# Autodesk Inventor assembly: Head
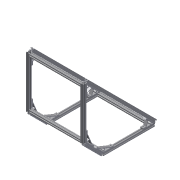
[picture p0: Inventor's stored thumbnail of the model, 180x180]
Saved by Autodesk Inventor 2014 SP1 (Build 180222100, 222)
## iProperties
Created: 2015-02-11
Part Number: Head
Document SubType Name: Assembly
Designer: Simen
Author: Simen
## Documents named in this file (6)
- C:\Users\Simen\Documents\git\Eit\skjellet\Head.iam
- C:\Users\Simen\Documents\git\Eit\skjellet\KHFS5_2020_350.ipt
- C:\Users\Simen\Documents\git\Eit\skjellet\HBL45TS6hbl45ts6.ipt
- C:\Users\Simen\Documents\git\Eit\skjellet\KHFS5_2020_660.ipt
- C:\Users\Simen\Documents\git\Eit\skjellet\HBL135TS6.iam
- C:\Users\Simen\Documents\git\Eit\skjellet\KHFS5_2020_165.ipt
## Components (20 placed, 3 different names)
1. HBL45TS6hbl45ts6:1 — Mate:1, Flush:1, Mate:2, Mate:23
2. KHFS5-2020-4000:1 — Mate:1, Flush:1, Mate:2, Flush:2, Angle:1, Mate:3, Mate:6, Flush:5, Mate:7, Mate:24, Flush:13, Flush:14, Mate:30, Flush:23, Flush:24
3. KHFS5-2020-4000:2 — Flush:2, Angle:1, Mate:3, Mate:21, Mate:22, Flush:12, Mate:23, Flush:22
4. HBL135TS6:1 [sub-assembly] — Mate:6, Flush:5, Mate:7
5. KHFS5-2020-4000:3 — Mate:24, Flush:13, Flush:14, Mate:25, Flush:15, Flush:16
6. KHFS5-2020-4000:4 — Mate:26, Flush:17, Flush:18, Mate:27, Flush:19, Flush:20
7. KHFS5-2020-4000:7 — Mate:25, Flush:15, Flush:16
8. HBL45TS6hbl45ts6:2
9. HBL135TS6:2 [sub-assembly] — Mate:31, Flush:27
10. KHFS5-2020-4000:8 — Mate:27, Flush:19, Flush:20, Flush:21
11. HBL45TS6hbl45ts6:3 — Mate:28
12. HBL135TS6:3 [sub-assembly] — Mate:32
13. KHFS5-2020-4000:9 — Mate:22, Flush:12, Mate:26, Flush:17, Flush:18, Mate:29, Flush:25, Flush:26
14. HBL45TS6hbl45ts6:4 — Mate:21
15. HBL135TS6:4 [sub-assembly] — Mate:33, Flush:28
16. KHFS5-2020-4000:10 — Flush:21, Mate:28, Flush:22
17. KHFS5-2020-4000:11 — Mate:30, Flush:23, Flush:24
18. KHFS5-2020-4000:12 — Mate:29, Flush:25, Flush:26
19. KHFS5-2020-4000:13 — Mate:31, Flush:27, Mate:32, Flush:29
20. KHFS5-2020-4000:14 — Mate:33, Flush:28, Flush:29
## Relationships (58: Mate 30, Flush 27, Angle 1)
- Mate:1: HBL45TS6hbl45ts6:1 ↔ KHFS5-2020-4000:1
- Flush:1: HBL45TS6hbl45ts6:1 ↔ KHFS5-2020-4000:1
- Mate:2: HBL45TS6hbl45ts6:1 ↔ KHFS5-2020-4000:1
- Flush:2: KHFS5-2020-4000:1 ↔ KHFS5-2020-4000:2
- Angle:1 (-45 deg): KHFS5-2020-4000:1 ↔ KHFS5-2020-4000:2
- Mate:3: KHFS5-2020-4000:1 ↔ KHFS5-2020-4000:2
- Mate:6: KHFS5-2020-4000:1 ↔ HBL135TS6:1
- Flush:5: KHFS5-2020-4000:1 ↔ HBL135TS6:1
- Mate:7: KHFS5-2020-4000:1 ↔ HBL135TS6:1
- [Mate]: KHFS5-2020-4000:7 ↔ HBL45TS6hbl45ts6:2
- [Flush]: KHFS5-2020-4000:7 ↔ HBL45TS6hbl45ts6:2
- [Mate]: KHFS5-2020-4000:7 ↔ HBL45TS6hbl45ts6:2
- [Mate]: KHFS5-2020-4000:7 ↔ HBL135TS6:2
- [Flush]: KHFS5-2020-4000:7 ↔ HBL135TS6:2
- [Mate]: KHFS5-2020-4000:7 ↔ HBL135TS6:2
- [Mate]: KHFS5-2020-4000:8 ↔ HBL45TS6hbl45ts6:3
- [Flush]: KHFS5-2020-4000:8 ↔ HBL45TS6hbl45ts6:3
- [Mate]: KHFS5-2020-4000:8 ↔ HBL45TS6hbl45ts6:3
- [Mate]: KHFS5-2020-4000:8 ↔ HBL135TS6:3
- [Flush]: KHFS5-2020-4000:8 ↔ HBL135TS6:3
- [Mate]: KHFS5-2020-4000:8 ↔ HBL135TS6:3
- [Mate]: KHFS5-2020-4000:9 ↔ HBL45TS6hbl45ts6:4
- [Flush]: KHFS5-2020-4000:9 ↔ HBL45TS6hbl45ts6:4
- [Mate]: KHFS5-2020-4000:9 ↔ HBL45TS6hbl45ts6:4
- [Mate]: KHFS5-2020-4000:9 ↔ HBL135TS6:4
- [Flush]: KHFS5-2020-4000:9 ↔ HBL135TS6:4
- [Mate]: KHFS5-2020-4000:9 ↔ HBL135TS6:4
- Mate:21: KHFS5-2020-4000:2 ↔ HBL45TS6hbl45ts6:4
- Mate:22: KHFS5-2020-4000:2 ↔ KHFS5-2020-4000:9
- Flush:12: KHFS5-2020-4000:2 ↔ KHFS5-2020-4000:9
- Mate:23: HBL45TS6hbl45ts6:1 ↔ KHFS5-2020-4000:2
- Mate:24: KHFS5-2020-4000:1 ↔ KHFS5-2020-4000:3
- Flush:13: KHFS5-2020-4000:1 ↔ KHFS5-2020-4000:3
- Flush:14: KHFS5-2020-4000:1 ↔ KHFS5-2020-4000:3
- Mate:25: KHFS5-2020-4000:3 ↔ KHFS5-2020-4000:7
- Flush:15: KHFS5-2020-4000:3 ↔ KHFS5-2020-4000:7
- Flush:16: KHFS5-2020-4000:3 ↔ KHFS5-2020-4000:7
- Mate:26: KHFS5-2020-4000:4 ↔ KHFS5-2020-4000:9
- Flush:17: KHFS5-2020-4000:4 ↔ KHFS5-2020-4000:9
- Flush:18: KHFS5-2020-4000:4 ↔ KHFS5-2020-4000:9
- Mate:27: KHFS5-2020-4000:4 ↔ KHFS5-2020-4000:8
- Flush:19: KHFS5-2020-4000:4 ↔ KHFS5-2020-4000:8
- Flush:20: KHFS5-2020-4000:4 ↔ KHFS5-2020-4000:8
- Flush:21: KHFS5-2020-4000:8 ↔ KHFS5-2020-4000:10
- Mate:28: HBL45TS6hbl45ts6:3 ↔ KHFS5-2020-4000:10
- Flush:22: KHFS5-2020-4000:2 ↔ KHFS5-2020-4000:10
- Mate:29: KHFS5-2020-4000:9 ↔ KHFS5-2020-4000:12
- Mate:30: KHFS5-2020-4000:1 ↔ KHFS5-2020-4000:11
- Flush:23: KHFS5-2020-4000:1 ↔ KHFS5-2020-4000:11
- Flush:24: KHFS5-2020-4000:1 ↔ KHFS5-2020-4000:11
- Flush:25: KHFS5-2020-4000:9 ↔ KHFS5-2020-4000:12
- Flush:26: KHFS5-2020-4000:9 ↔ KHFS5-2020-4000:12
- Mate:31: HBL135TS6:2 ↔ KHFS5-2020-4000:13
- Flush:27: HBL135TS6:2 ↔ KHFS5-2020-4000:13
- Mate:32: HBL135TS6:3 ↔ KHFS5-2020-4000:13
- Mate:33: HBL135TS6:4 ↔ KHFS5-2020-4000:14
- Flush:28: HBL135TS6:4 ↔ KHFS5-2020-4000:14
- Flush:29: KHFS5-2020-4000:13 ↔ KHFS5-2020-4000:14
## Named parameters: d13_d0 = 0 mm, d14_d1 = 0 mm, d15_d2 = 0 mm, d16_d10 = 0 mm, d17_d11 = 0 mm, d18_d12 = 0 mm, d19_d0 = 0 mm, d20_d1 = 0 mm, d21_d2 = 0 mm, d22_d10 = 0 mm, d23_d11 = 0 mm, d24_d12 = 0 mm, d25_d0 = 0 mm, d26_d1 = 0 mm, d27_d2 = 0 mm, d28_d10 = 0 mm, d29_d11 = 0 mm, d30_d12 = 0 mm
